# Autodesk Inventor assembly: xDriveShaftFront
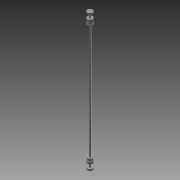
[picture p0: Inventor's stored thumbnail of the model, 180x180]
Saved by Autodesk Inventor 2013 (Build 170138000, 138)
## iProperties
Created: 2015-01-14
Part Number: xDriveShaftFront
Document SubType Name: Assembly
Designer: dzban
Author: dzban
## Documents named in this file (4)
- D:\PIRX\Artisan\OPENSOURCE\SmallPieces\xDriveShaftFront.iam
- D:\PIRX\Artisan\OPENSOURCE\StockComponents\625ZZ_bearing.ipt
- D:\PIRX\Artisan\OPENSOURCE\StockComponents\gt2_20_pulley.ipt
- D:\PIRX\Artisan\OPENSOURCE\SmallPieces\xDriveShaft.ipt
## Components (5 placed, 3 different names)
1. 625ZZ_bearing:1 — Insert:2, Insert:3
2. 625ZZ_bearing:2 — Insert:1, Insert:4
3. gt2_20_pulley:1 — Insert:4
4. gt2_20_pulley:2 — Insert:3
5. xDriveShaft:1 — Insert:1, Insert:2
## Relationships (4: Insert 4)
- Insert:1 (-5 mm): 625ZZ_bearing:2 ↔ xDriveShaft:1
- Insert:2 (-5 mm): 625ZZ_bearing:1 ↔ xDriveShaft:1
- Insert:3 (-32 mm): 625ZZ_bearing:1 ↔ gt2_20_pulley:2
- Insert:4 (-32 mm): 625ZZ_bearing:2 ↔ gt2_20_pulley:1
